# Autodesk Inventor assembly: 脚四半
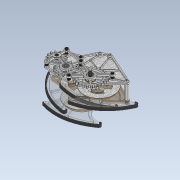
[picture p0: Inventor's stored thumbnail of the model, 180x180]
Saved by Autodesk Inventor 2020.2 (Build 242310000, 310)
## iProperties
Created: 2020-03-11
Part Number: 脚四半
Document SubType Name: Assembly
Designer: aoyam
Mass: 216.07 g
Surface Area: 1653.51 cm^2
Volume: 107.747 cm^3
Density: 2.00533 g/cm^3
Author: aoyam
## Documents named in this file (37)
- C:\Users\aoyam\Desktop\SRDC_local\Inventor\二年機\Geminiβ\脚\脚四半.iam
- C:\Users\aoyam\Desktop\SRDC_local\Inventor\二年機\Geminiβ\汎用部品\ワッシャD8d6m0.5.ipt
- C:\Users\aoyam\Desktop\SRDC_local\Inventor\二年機\Geminiβ\汎用部品\ワッシャD7d4m0.5.ipt
- C:\Users\aoyam\Desktop\SRDC_local\Inventor\二年機\Geminiβ\汎用部品\ｍ2歯数17ギアd3.99.ipt
- C:\Users\aoyam\Desktop\SRDC_local\Inventor\二年機\Geminiβ\汎用部品\スペーサーM3L30アルミ.ipt
- C:\Users\aoyam\Desktop\SRDC_local\Inventor\二年機\Geminiβ\汎用部品\ネジボタンM3L6.ipt
- C:\Users\aoyam\Desktop\SRDC_local\Inventor\二年機\Geminiβ\汎用部品\ネジボタンM3L8.ipt
- C:\Users\aoyam\Desktop\SRDC_local\Inventor\二年機\Geminiβ\汎用部品\スペーサーM3L30樹脂.ipt
- C:\Users\aoyam\Desktop\SRDC_local\Inventor\二年機\Geminiβ\汎用部品\オイレスFd6D8L7.ipt
- C:\Users\aoyam\Desktop\SRDC_local\Inventor\二年機\Geminiβ\汎用部品\ネジアルミM3L6.ipt
- C:\Users\aoyam\Desktop\SRDC_local\Inventor\二年機\Geminiβ\脚\脚フレーム外側後.ipt
- C:\Users\aoyam\Desktop\SRDC_local\Inventor\二年機\Geminiβ\脚\ネジクランク\脚一枚.iam
- C:\Users\aoyam\Desktop\SRDC_local\Inventor\二年機\Geminiβ\脚\ネジクランク\カムL4F.ipt
- C:\Users\aoyam\Desktop\SRDC_local\Inventor\二年機\Geminiβ\汎用部品\オイレスドライメットFd10D12L3.ipt
- C:\Users\aoyam\Desktop\SRDC_local\Inventor\二年機\Geminiβ\汎用部品\ｍ2歯数25ギアネジ.ipt
- C:\Users\aoyam\Desktop\SRDC_local\Inventor\二年機\Geminiβ\汎用部品\オイレスドライメットFd10D12L4.ipt
- C:\Users\aoyam\Desktop\SRDC_local\Inventor\二年機\Geminiβ\脚\ネジクランク\カムL3.ipt
- C:\Users\aoyam\Desktop\SRDC_local\Inventor\二年機\Geminiβ\脚\ネジクランク\カムL4.ipt
- C:\Users\aoyam\Desktop\SRDC_local\Inventor\二年機\Geminiβ\汎用部品\ネジキャップM3L45.ipt
- C:\Users\aoyam\Desktop\SRDC_local\Inventor\二年機\Geminiβ\汎用部品\ナットナイロンM3.ipt
- C:\Users\aoyam\Desktop\SRDC_local\Inventor\二年機\Geminiβ\汎用部品\スペーサーM3L40アルミ.ipt
- C:\Users\aoyam\Desktop\SRDC_local\Inventor\二年機\Geminiβ\汎用部品\ネジ超極低頭M3L4.ipt
- C:\Users\aoyam\Desktop\SRDC_local\Inventor\二年機\Geminiβ\脚\脚フレーム内側後改.ipt
- C:\Users\aoyam\Desktop\SRDC_local\Inventor\二年機\Geminiβ\汎用部品\ベアリングFd4D11B4.ipt
- C:\Users\aoyam\Desktop\SRDC_local\Inventor\二年機\Geminiβ\汎用部品\ネジ皿M3L8.ipt
- C:\Users\aoyam\Desktop\SRDC_local\Inventor\二年機\Geminiβ\汎用部品\ベアリングFd6D12B4.ipt
- C:\Users\aoyam\Desktop\SRDC_local\Inventor\二年機\Geminiβ\汎用部品\ｍ2歯数14ギアd12.ipt
- C:\Users\aoyam\Desktop\SRDC_local\Inventor\二年機\Geminiβ\汎用部品\オイレスFd6D8L4.ipt
- C:\Users\aoyam\Desktop\SRDC_local\Inventor\二年機\Geminiβ\脚\脚ギアトレイン2.ipt
- C:\Users\aoyam\Desktop\SRDC_local\Inventor\二年機\Geminiβ\汎用部品\ワッシャD10d6m0.3.ipt
- C:\Users\aoyam\Desktop\SRDC_local\Inventor\二年機\Geminiβ\汎用部品\オイレス外径8内径6L3.ipt
- C:\Users\aoyam\Desktop\SRDC_local\Inventor\二年機\Geminiβ\汎用部品\ポリスラd6D14t0.25.ipt
- C:\Users\aoyam\Desktop\SRDC_local\Inventor\二年機\Geminiβ\汎用部品\スペーサー中空M3L5樹脂.ipt
- C:\Users\aoyam\Desktop\SRDC_local\Inventor\二年機\Geminiβ\汎用部品\ネジボタンM3L10.ipt
- C:\Users\aoyam\Desktop\SRDC_local\Inventor\二年機\Geminiβ\汎用部品\平行ピンD4L12.ipt
- C:\Users\aoyam\Desktop\SRDC_local\Inventor\二年機\Geminiβ\汎用部品\スペーサー中空M3L4樹脂.ipt
- C:\Users\aoyam\Desktop\SRDC_local\Inventor\二年機\Geminiβ\汎用部品\ネジキャップM3L15.ipt
## Components (61 placed, 36 different names)
1. ワッシャD7d4m0.5:1 — 挿入:9, 挿入:169
2. ｍ2歯数17ギアd3.99:1 — 挿入:9, 挿入:11
3. ワッシャD7d4m0.5:2 — 挿入:11, 挿入:155
4. ワッシャD8d6m0.5:2 — 挿入:160, 挿入:161
5. スペーサーM3L30アルミ:1 — 挿入:93, メイト:9, メイト:10, メイト:11, メイト:12
6. ネジボタンM3L6:1 — 挿入:148
7. ネジボタンM3L8:4 — 挿入:97
8. スペーサーM3L30樹脂:1 — 挿入:146, 挿入:151
9. スペーサーM3L30樹脂:2 — 挿入:152, 挿入:153
10. オイレスFd6D8L7:1 — 挿入:136, 挿入:137
11. オイレスFd6D8L7:2 — 挿入:134
12. オイレスFd6D8L7:3 — 挿入:135
13. オイレスFd6D8L7:4 — 挿入:133, 挿入:139
14. ワッシャD8d6m0.5:3 — 挿入:93, 挿入:129
15. ワッシャD8d6m0.5:4 — 挿入:130, 挿入:138
16. ワッシャD8d6m0.5:5 — 挿入:129, 挿入:139
17. ネジアルミM3L6:1 — 挿入:147
18. ネジアルミM3L6:2 — 挿入:149
19. ネジアルミM3L6:3 — 挿入:98
20. ネジアルミM3L6:4 — 挿入:99
21. 脚フレーム外側後:1 — 挿入:97, 挿入:98, 挿入:99, メイト:1, 挿入:111, 挿入:124, 挿入:138, 挿入:151, 挿入:153
22. 脚一枚:1 [sub-assembly] — 挿入:103, 挿入:104, メイト:1, 挿入:109, 挿入:110, メイト:9, 挿入:136
23. 脚一枚:2 [sub-assembly] — 挿入:103, 挿入:104, 挿入:105, 挿入:106, メイト:10, 挿入:135
24. 脚一枚:3 [sub-assembly] — 挿入:105, 挿入:106, 挿入:107, 挿入:108, メイト:11, 挿入:134
25. 脚一枚:4 [sub-assembly] — 挿入:107, 挿入:108, メイト:6, メイト:7, メイト:12, 挿入:133
26. カムL4F:1 — 挿入:109, 挿入:110, 挿入:111, 挿入:112, 挿入:119, 挿入:120
27. オイレスドライメットFd10D12L3:1 — 挿入:112
28. ｍ2歯数25ギアネジ:1 — 挿入:114, 挿入:115, 挿入:116, メイト:6, メイト:13, メイト:14, 挿入:164
29. オイレスドライメットFd10D12L3:2 — 挿入:114, 挿入:165
30. カムL3:1 — 挿入:115, 挿入:116, 挿入:121, 挿入:122, メイト:13
31. オイレスドライメットFd10D12L4:1 — 挿入:118, 挿入:150, 挿入:164
32. カムL4:1 — 挿入:118, メイト:7
33. ネジキャップM3L45:1 — 挿入:119, メイト:14
34. ネジキャップM3L45:2 — 挿入:120
35. ナットナイロンM3:1 — 挿入:121, メイト:8
36. ナットナイロンM3:2 — 挿入:122, メイト:8
37. スペーサーM3L40アルミ:1 — 挿入:124, 挿入:127, 挿入:181
38. ネジ超極低頭M3L4:1 — 挿入:127
39. ワッシャD8d6m0.5:6 — 挿入:130, 挿入:137
40. 脚フレーム内側後改:1 — 挿入:146, 挿入:147, 挿入:148, 挿入:149, 挿入:150, 挿入:152, 挿入:154, 挿入:157, 挿入:163, 挿入:173, 挿入:174, 挿入:175, 挿入:176
41. ベアリングFd4D11B4:1 — 挿入:154, 挿入:155
42. ベアリングFd4D11B4:2 — 挿入:168, 挿入:169, 挿入:180
43. ネジ皿M3L8:1 — 挿入:157
44. ベアリングFd6D12B4:1 — 挿入:159, 挿入:161, 挿入:167
45. ｍ2歯数14ギアd12:1 — 挿入:159
46. オイレスFd6D8L4:1 — 挿入:160, 挿入:163
47. 脚ギアトレイン2:1 — 挿入:165, 挿入:168, 挿入:170, 挿入:177, 挿入:178, 挿入:179, 挿入:182
48. ワッシャD10d6m0.3:1 — 挿入:167
49. オイレス外径8内径6L3:1 — 挿入:170, 挿入:172
50. ポリスラd6D14t0.25:1 — 挿入:171, 挿入:172
51. ポリスラd6D14t0.25:2 — 挿入:171
52. スペーサー中空M3L5樹脂:1 — 挿入:173
53. スペーサー中空M3L5樹脂:2 — 挿入:174
54. スペーサー中空M3L5樹脂:3 — 挿入:175
55. スペーサー中空M3L5樹脂:4 — 挿入:176
56. ネジボタンM3L10:1 — 挿入:177
57. ネジボタンM3L10:2 — 挿入:178
58. ネジボタンM3L10:3 — 挿入:179
59. 平行ピンD4L12:1 — 挿入:180
60. スペーサー中空M3L4樹脂:1 — 挿入:181
61. ネジキャップM3L15:1 — 挿入:182
## Relationships (78: Insert 68, Mate 10)
- 挿入:9 [Insert]: ワッシャD7d4m0.5:1 ↔ ｍ2歯数17ギアd3.99:1
- 挿入:11 [Insert]: ｍ2歯数17ギアd3.99:1 ↔ ワッシャD7d4m0.5:2
- 挿入:93 [Insert]: スペーサーM3L30アルミ:1 ↔ ワッシャD8d6m0.5:3
- 挿入:97 [Insert]: ネジボタンM3L8:4 ↔ 脚フレーム外側後:1
- 挿入:98 [Insert]: ネジアルミM3L6:3 ↔ 脚フレーム外側後:1
- 挿入:99 [Insert]: ネジアルミM3L6:4 ↔ 脚フレーム外側後:1
- 挿入:103 [Insert]: 脚一枚:1 ↔ 脚一枚:2
- 挿入:104 [Insert]: 脚一枚:1 ↔ 脚一枚:2
- 挿入:105 [Insert]: 脚一枚:2 ↔ 脚一枚:3
- 挿入:106 [Insert]: 脚一枚:2 ↔ 脚一枚:3
- 挿入:107 [Insert]: 脚一枚:3 ↔ 脚一枚:4
- 挿入:108 [Insert]: 脚一枚:3 ↔ 脚一枚:4
- メイト:1 [Mate] (1 mm): 脚フレーム外側後:1 ↔ 脚一枚:1
- 挿入:109 [Insert]: 脚一枚:1 ↔ カムL4F:1
- 挿入:110 [Insert]: 脚一枚:1 ↔ カムL4F:1
- 挿入:111 [Insert]: 脚フレーム外側後:1 ↔ カムL4F:1
- 挿入:112 [Insert]: カムL4F:1 ↔ オイレスドライメットFd10D12L3:1
- 挿入:114 [Insert]: ｍ2歯数25ギアネジ:1 ↔ オイレスドライメットFd10D12L3:2
- 挿入:115 [Insert]: ｍ2歯数25ギアネジ:1 ↔ カムL3:1
- 挿入:116 [Insert]: ｍ2歯数25ギアネジ:1 ↔ カムL3:1
- メイト:6 [Mate]: 脚一枚:4 ↔ ｍ2歯数25ギアネジ:1
- 挿入:118 [Insert]: オイレスドライメットFd10D12L4:1 ↔ カムL4:1
- メイト:7 [Mate]: 脚一枚:4 ↔ カムL4:1
- 挿入:119 [Insert]: カムL4F:1 ↔ ネジキャップM3L45:1
- 挿入:120 [Insert]: カムL4F:1 ↔ ネジキャップM3L45:2
- 挿入:121 [Insert]: カムL3:1 ↔ ナットナイロンM3:1
- 挿入:122 [Insert]: カムL3:1 ↔ ナットナイロンM3:2
- メイト:8 [Mate]: ナットナイロンM3:1 ↔ ナットナイロンM3:2
- 挿入:124 [Insert] (3 mm): 脚フレーム外側後:1 ↔ スペーサーM3L40アルミ:1
- 挿入:127 [Insert]: スペーサーM3L40アルミ:1 ↔ ネジ超極低頭M3L4:1
- 挿入:129 [Insert]: ワッシャD8d6m0.5:3 ↔ ワッシャD8d6m0.5:5
- 挿入:130 [Insert]: ワッシャD8d6m0.5:4 ↔ ワッシャD8d6m0.5:6
- メイト:9 [Mate]: スペーサーM3L30アルミ:1 ↔ 脚一枚:1
- メイト:10 [Mate]: スペーサーM3L30アルミ:1 ↔ 脚一枚:2
- メイト:11 [Mate]: スペーサーM3L30アルミ:1 ↔ 脚一枚:3
- メイト:12 [Mate]: スペーサーM3L30アルミ:1 ↔ 脚一枚:4
- 挿入:133 [Insert]: オイレスFd6D8L7:4 ↔ 脚一枚:4
- 挿入:134 [Insert]: オイレスFd6D8L7:2 ↔ 脚一枚:3
- 挿入:135 [Insert]: オイレスFd6D8L7:3 ↔ 脚一枚:2
- 挿入:136 [Insert]: オイレスFd6D8L7:1 ↔ 脚一枚:1
- 挿入:137 [Insert]: オイレスFd6D8L7:1 ↔ ワッシャD8d6m0.5:6
- 挿入:138 [Insert]: ワッシャD8d6m0.5:4 ↔ 脚フレーム外側後:1
- 挿入:139 [Insert]: オイレスFd6D8L7:4 ↔ ワッシャD8d6m0.5:5
- メイト:13 [Mate]: ｍ2歯数25ギアネジ:1 ↔ カムL3:1
- 挿入:146 [Insert]: スペーサーM3L30樹脂:1 ↔ 脚フレーム内側後改:1
- 挿入:147 [Insert]: ネジアルミM3L6:1 ↔ 脚フレーム内側後改:1
- 挿入:148 [Insert]: ネジボタンM3L6:1 ↔ 脚フレーム内側後改:1
- 挿入:149 [Insert]: ネジアルミM3L6:2 ↔ 脚フレーム内側後改:1
- 挿入:150 [Insert]: オイレスドライメットFd10D12L4:1 ↔ 脚フレーム内側後改:1
- メイト:14 [Mate]: ｍ2歯数25ギアネジ:1 ↔ ネジキャップM3L45:1
- 挿入:151 [Insert]: スペーサーM3L30樹脂:1 ↔ 脚フレーム外側後:1
- 挿入:152 [Insert]: スペーサーM3L30樹脂:2 ↔ 脚フレーム内側後改:1
- 挿入:153 [Insert]: スペーサーM3L30樹脂:2 ↔ 脚フレーム外側後:1
- 挿入:154 [Insert]: 脚フレーム内側後改:1 ↔ ベアリングFd4D11B4:1
- 挿入:155 [Insert]: ワッシャD7d4m0.5:2 ↔ ベアリングFd4D11B4:1
- 挿入:157 [Insert]: 脚フレーム内側後改:1 ↔ ネジ皿M3L8:1
- 挿入:159 [Insert]: ベアリングFd6D12B4:1 ↔ ｍ2歯数14ギアd12:1
- 挿入:160 [Insert]: ワッシャD8d6m0.5:2 ↔ オイレスFd6D8L4:1
- 挿入:161 [Insert]: ワッシャD8d6m0.5:2 ↔ ベアリングFd6D12B4:1
- 挿入:163 [Insert]: 脚フレーム内側後改:1 ↔ オイレスFd6D8L4:1
- 挿入:164 [Insert]: ｍ2歯数25ギアネジ:1 ↔ オイレスドライメットFd10D12L4:1
- 挿入:165 [Insert]: オイレスドライメットFd10D12L3:2 ↔ 脚ギアトレイン2:1
- 挿入:167 [Insert]: ベアリングFd6D12B4:1 ↔ ワッシャD10d6m0.3:1
- 挿入:168 [Insert]: ベアリングFd4D11B4:2 ↔ 脚ギアトレイン2:1
- 挿入:169 [Insert]: ワッシャD7d4m0.5:1 ↔ ベアリングFd4D11B4:2
- 挿入:170 [Insert]: 脚ギアトレイン2:1 ↔ オイレス外径8内径6L3:1
- 挿入:171 [Insert]: ポリスラd6D14t0.25:1 ↔ ポリスラd6D14t0.25:2
- 挿入:172 [Insert]: オイレス外径8内径6L3:1 ↔ ポリスラd6D14t0.25:1
- 挿入:173 [Insert]: 脚フレーム内側後改:1 ↔ スペーサー中空M3L5樹脂:1
- 挿入:174 [Insert]: 脚フレーム内側後改:1 ↔ スペーサー中空M3L5樹脂:2
- 挿入:175 [Insert]: 脚フレーム内側後改:1 ↔ スペーサー中空M3L5樹脂:3
- 挿入:176 [Insert]: 脚フレーム内側後改:1 ↔ スペーサー中空M3L5樹脂:4
- 挿入:177 [Insert]: 脚ギアトレイン2:1 ↔ ネジボタンM3L10:1
- 挿入:178 [Insert]: 脚ギアトレイン2:1 ↔ ネジボタンM3L10:2
- 挿入:179 [Insert]: 脚ギアトレイン2:1 ↔ ネジボタンM3L10:3
- 挿入:180 [Insert]: ベアリングFd4D11B4:2 ↔ 平行ピンD4L12:1
- 挿入:181 [Insert]: スペーサーM3L40アルミ:1 ↔ スペーサー中空M3L4樹脂:1
- 挿入:182 [Insert]: 脚ギアトレイン2:1 ↔ ネジキャップM3L15:1
